# Autodesk Inventor assembly: AM14U3 Long Frame Half
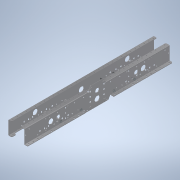
[picture p0: Inventor's stored thumbnail of the model, 180x180]
Saved by Autodesk Inventor 2020 (Build 240168000, 168)
## iProperties
Created: 2015-12-05
Part Number: AM14U3 Long Frame Half
Document SubType Name: Assembly
Designer: PhillipD
Author: PhillipD
Revision Number: ANY
## Documents named in this file (5)
- C:\Users\srini\Documents\FRC\2020\2018_KOP\Inventor\FRC 2018 Drive Base Inventor\FIRST 2018 Drive Base\Parts\AM14U3 Long Frame Half.iam
- C:\Users\srini\Documents\FRC\2020\2018_KOP\Inventor\FRC 2018 Drive Base Inventor\FIRST 2018 Drive Base\Parts\Churro 3375.ipt
- C:\Users\srini\Documents\FRC\2020\2018_KOP\Inventor\FRC 2018 Drive Base Inventor\FIRST 2018 Drive Base\Parts\FHTS 0.25-20-0.75_FHTS 0.25-20-G-0.75-C.ipt
- C:\Users\srini\Documents\FRC\2020\2018_KOP\Inventor\FRC 2018 Drive Base Inventor\FIRST 2018 Drive Base\Parts\AM14U3 Inside Sheet Rev2.ipt
- C:\Users\srini\Documents\FRC\2020\2018_KOP\Inventor\FRC 2018 Drive Base Inventor\FIRST 2018 Drive Base\Parts\AM14U3 Outside Sheet Rev1_DefaultSM-FLAT-PATTERN.ipt
## Components (13 placed, 11 different names)
1. Churro 3375_120
2. Churro 3375_121
3. FHTS 0.25-20-0.75_FHTS 0.25-20-G-0.75-C_125
4. FHTS 0.25-20-0.75_FHTS 0.25-20-G-0.75-C_126
5. FHTS 0.25-20-0.75_FHTS 0.25-20-G-0.75-C_127
6. FHTS 0.25-20-0.75_FHTS 0.25-20-G-0.75-C_128
7. FHTS 0.25-20-0.75_FHTS 0.25-20-G-0.75-C_129
8. FHTS 0.25-20-0.75_FHTS 0.25-20-G-0.75-C_130
9. AM14U3 Inside Sheet Rev2_136
10. AM14U3 Outside Sheet Rev1_DefaultSM-FLAT-PATTERN_137 — Insert:1, Insert:2, Insert:3
11. FHTS 0.25-20-0.75_FHTS 0.25-20-G-0.75-C:9 — Insert:1
12. FHTS 0.25-20-0.75_FHTS 0.25-20-G-0.75-C:10 — Insert:2
13. FHTS 0.25-20-0.75_FHTS 0.25-20-G-0.75-C:11 — Insert:3
## Relationships (3: Insert 3)
- Insert:1: AM14U3 Outside Sheet Rev1_DefaultSM-FLAT-PATTERN_137 ↔ FHTS 0.25-20-0.75_FHTS 0.25-20-G-0.75-C:9
- Insert:2: AM14U3 Outside Sheet Rev1_DefaultSM-FLAT-PATTERN_137 ↔ FHTS 0.25-20-0.75_FHTS 0.25-20-G-0.75-C:10
- Insert:3: AM14U3 Outside Sheet Rev1_DefaultSM-FLAT-PATTERN_137 ↔ FHTS 0.25-20-0.75_FHTS 0.25-20-G-0.75-C:11
